# Autodesk Inventor assembly: Frame Test V3
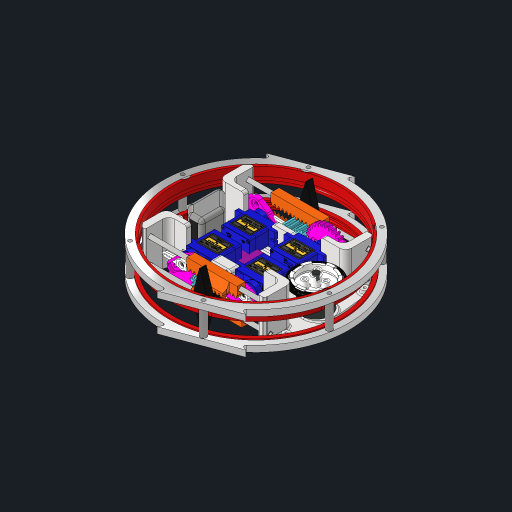
[picture p0: Inventor's stored thumbnail of the model, 512x512]
Saved by Autodesk Inventor 2023.2 (Build 272271030, 271C)
## iProperties
Created: 2024-01-27
Part Number: Frame Test V3
Document SubType Name: Assembly
Designer: robpl
Author: robpl
## Documents named in this file (17)
- C:\Users\robpl\OneDrive\Documents\Arduino\Onslaught\CAD\Onslaught V1.iam
- C:\Users\robpl\OneDrive\Documents\Arduino\Onslaught\CAD\Frame.ipt
- C:\Users\robpl\OneDrive\Documents\Arduino\Onslaught\CAD\SG90 - Micro Servo 9g - Tower Pro\SG90 - Micro Servo 9g - Tower Pro.ipt
- C:\Users\robpl\OneDrive\Documents\Arduino\Onslaught\CAD\802035 Battery.ipt
- C:\Users\robpl\OneDrive\Documents\Arduino\Onslaught\CAD\Ar620.ipt
- C:\Users\robpl\OneDrive\Documents\Arduino\Onslaught\CAD\Emax 1806 2280kv.ipt
- C:\Users\robpl\OneDrive\Documents\Arduino\Onslaught\CAD\BLHeli 12A ESC.ipt
- C:\Users\robpl\OneDrive\Documents\Arduino\Onslaught\CAD\Frame Test\Frame Test V3\Design Accelerator\Spur Gears3.iam
- C:\Users\robpl\OneDrive\Documents\Arduino\Onslaught\CAD\Frame Test\Servo Gear v3.ipt
- C:\Users\robpl\OneDrive\Documents\Arduino\Onslaught\CAD\Frame Test\Idler Gear.ipt
- C:\Users\robpl\OneDrive\Documents\Arduino\Onslaught\CAD\Frame Test\Rail.ipt
- C:\Users\robpl\OneDrive\Documents\Arduino\Onslaught\CAD\Frame Test\Rack V3.ipt
- C:\Users\robpl\OneDrive\Documents\Arduino\Onslaught\CAD\Frame Test\Leg V3.ipt
- C:\Users\robpl\OneDrive\Documents\Arduino\Onslaught\CAD\tamiya-slim-tire-set-1.snapshot.2\36mm Slim Tamiya.iam
- C:\Users\robpl\OneDrive\Documents\Arduino\Onslaught\CAD\2x6x2.5mm Bearing.ipt
- C:\Users\robpl\OneDrive\Documents\Arduino\Onslaught\CAD\Bearing Spacer.ipt
- C:\Users\robpl\OneDrive\Documents\Arduino\Onslaught\CAD\Frame Test\Ring.iam
## Components (35 placed, 16 different names)
1. Frame:1 — Mate:2, Mate:3, Mate:4, Mate:5, Mate:6, Mate:8, Mate:12, Mate:15, Mate:16, Mate:25, Angle:1, Angle:2, Angle:3, Angle:4, Flush:13, Flush:14, Mate:53, Mate:54, Mate:55, Mate:56, Mate:57, Mate:58, Mate:59, Mate:60, Mate:61, Mate:62, Mate:63, Mate:64, Flush:19, Flush:20, Mate:67, Mate:68, Flush:21, Mate:69, Mate:73, Mate:74, Mate:75, Mate:76, Flush:22, Mate:78, Mate:79, Mate:80, Mate:81, Mate:82, Mate:83, Mate:85
2. SG90 - Micro Servo 9g - Tower Pro:1 — Mate:15, Mate:16, Mate:29, Mate:32, Mate:55
3. SG90 - Micro Servo 9g - Tower Pro:2 — Mate:2, Mate:3, Mate:30, Mate:31, Mate:56, Mate:84
4. SG90 - Micro Servo 9g - Tower Pro:3 — Mate:4, Mate:8, Flush:10, Mate:24, Mate:54
5. SG90 - Micro Servo 9g - Tower Pro:4 — Mate:5, Mate:6, Mate:23, Flush:9, Mate:27, Mate:28, Mate:53
6. 802035 Battery:1 — Flush:6
7. 802035 Battery:2 — Flush:6
8. Ar620:1 — Mate:67, Mate:68, Flush:21
9. Emax 1806 2280kv:1 — Mate:12, Mate:21, Mate:65, Mate:66, Mate:82
10. BLHeli 12A ESC:1 — Mate:79
11. Spur Gears:2 [sub-assembly] — Mate:23, Flush:9
12. Servo Gear v3:1 — Flush:10, Mate:24
13. Idler Gear:1 — Mate:25, Flush:16
14. Servo Gear v3:2 — Mate:30, Mate:31
15. Servo Gear v3:3 — Mate:27, Mate:28
16. Servo Gear v3:4 — Mate:29, Mate:32
17. Rail:1 — Angle:1, Flush:14, Mate:62
18. Rail:2 — Angle:2, Flush:13, Mate:61
19. Rail:3 — Angle:4, Mate:63, Flush:19
20. Rail:4 — Angle:3, Mate:64, Flush:20
21. Rack V3:1 — Flush:18, Mate:51, Mate:52, Mate:58
22. Rack V3:2 — Flush:17, Mate:49, Mate:50, Mate:60
23. Rack V3:3 — Flush:17, Mate:59
24. Idler Gear:2 — Flush:16, Mate:85
25. Idler Gear:3 — Flush:15
26. Idler Gear:4 — Flush:15, Mate:83, Mate:84
27. Rack V3:4 — Flush:18, Mate:57
28. Leg V3:1 — Mate:49, Mate:50
29. Leg V3:2 — Mate:51, Mate:52
30. 36mm Slim Tamiya:1 [sub-assembly] — Mate:65, Mate:66
31. 2x6x2.5mm Bearing:1 — Mate:70, Mate:71
32. Bearing Spacer:1 — Mate:69, Mate:70, Mate:71, Mate:80, Mate:81
33. 2x6x2.5mm Bearing:2 — Mate:73, Mate:76
34. 2x6x2.5mm Bearing:3 — Mate:74, Mate:75
35. Ring:1 [sub-assembly] — Flush:22, Mate:78
## Relationships (71: Mate 54, Flush 13, Angle 4)
- Flush:6: 802035 Battery:1 ↔ 802035 Battery:2
- Mate:2: Frame:1 ↔ SG90 - Micro Servo 9g - Tower Pro:2
- Mate:3: Frame:1 ↔ SG90 - Micro Servo 9g - Tower Pro:2
- Mate:4: Frame:1 ↔ SG90 - Micro Servo 9g - Tower Pro:3
- Mate:5: Frame:1 ↔ SG90 - Micro Servo 9g - Tower Pro:4
- Mate:6: Frame:1 ↔ SG90 - Micro Servo 9g - Tower Pro:4
- Mate:8: Frame:1 ↔ SG90 - Micro Servo 9g - Tower Pro:3
- Mate:12 (1 mm): Frame:1 ↔ Emax 1806 2280kv:1
- Mate:15: Frame:1 ↔ SG90 - Micro Servo 9g - Tower Pro:1
- Mate:16: Frame:1 ↔ SG90 - Micro Servo 9g - Tower Pro:1
- Mate:21: Emax 1806 2280kv:1
- Mate:23: SG90 - Micro Servo 9g - Tower Pro:4 ↔ Spur Gears:2
- Flush:9: SG90 - Micro Servo 9g - Tower Pro:4 ↔ Spur Gears:2
- Flush:10: SG90 - Micro Servo 9g - Tower Pro:3 ↔ Servo Gear v3:1
- Mate:24: SG90 - Micro Servo 9g - Tower Pro:3 ↔ Servo Gear v3:1
- Mate:25: Frame:1 ↔ Idler Gear:1
- Mate:27: SG90 - Micro Servo 9g - Tower Pro:4 ↔ Servo Gear v3:3
- Mate:28: SG90 - Micro Servo 9g - Tower Pro:4 ↔ Servo Gear v3:3
- Mate:29: SG90 - Micro Servo 9g - Tower Pro:1 ↔ Servo Gear v3:4
- Mate:30: SG90 - Micro Servo 9g - Tower Pro:2 ↔ Servo Gear v3:2
- Mate:31: SG90 - Micro Servo 9g - Tower Pro:2 ↔ Servo Gear v3:2
- Mate:32: SG90 - Micro Servo 9g - Tower Pro:1 ↔ Servo Gear v3:4
- Angle:1 (0 deg): Frame:1 ↔ Rail:1
- Angle:2 (0 deg): Frame:1 ↔ Rail:2
- Angle:3 (0 deg): Frame:1 ↔ Rail:4
- Angle:4 (0 deg): Frame:1 ↔ Rail:3
- Flush:13: Frame:1 ↔ Rail:2
- Flush:14: Frame:1 ↔ Rail:1
- Flush:15: Idler Gear:3 ↔ Idler Gear:4
- Flush:16: Idler Gear:1 ↔ Idler Gear:2
- Flush:17: Rack V3:2 ↔ Rack V3:3
- Flush:18: Rack V3:1 ↔ Rack V3:4
- Mate:49 (-4.75 mm): Rack V3:2 ↔ Leg V3:1
- Mate:50 (-13.5 mm): Rack V3:2 ↔ Leg V3:1
- Mate:51 (-4.75 mm): Rack V3:1 ↔ Leg V3:2
- Mate:52 (-13.5 mm): Rack V3:1 ↔ Leg V3:2
- Mate:53: Frame:1 ↔ SG90 - Micro Servo 9g - Tower Pro:4
- Mate:54: Frame:1 ↔ SG90 - Micro Servo 9g - Tower Pro:3
- Mate:55: Frame:1 ↔ SG90 - Micro Servo 9g - Tower Pro:1
- Mate:56: Frame:1 ↔ SG90 - Micro Servo 9g - Tower Pro:2
- Mate:57: Frame:1 ↔ Rack V3:4
- Mate:58: Frame:1 ↔ Rack V3:1
- Mate:59: Frame:1 ↔ Rack V3:3
- Mate:60: Frame:1 ↔ Rack V3:2
- Mate:61: Frame:1 ↔ Rail:2
- Mate:62: Frame:1 ↔ Rail:1
- Mate:63: Frame:1 ↔ Rail:3
- Mate:64: Frame:1 ↔ Rail:4
- Flush:19: Frame:1 ↔ Rail:3
- Flush:20: Frame:1 ↔ Rail:4
- Mate:65: Emax 1806 2280kv:1 ↔ 36mm Slim Tamiya:1
- Mate:66: Emax 1806 2280kv:1 ↔ 36mm Slim Tamiya:1
- Mate:67: Frame:1 ↔ Ar620:1
- Mate:68: Frame:1 ↔ Ar620:1
- Flush:21: Frame:1 ↔ Ar620:1
- Mate:69: Frame:1 ↔ Bearing Spacer:1
- Mate:70: 2x6x2.5mm Bearing:1 ↔ Bearing Spacer:1
- Mate:71: 2x6x2.5mm Bearing:1 ↔ Bearing Spacer:1
- Mate:73: Frame:1 ↔ 2x6x2.5mm Bearing:2
- Mate:74: Frame:1 ↔ 2x6x2.5mm Bearing:3
- Mate:75: Frame:1 ↔ 2x6x2.5mm Bearing:3
- Mate:76: Frame:1 ↔ 2x6x2.5mm Bearing:2
- Flush:22 (-2.5 mm): Frame:1 ↔ Ring:1
- Mate:78: Frame:1 ↔ Ring:1
- Mate:79: Frame:1 ↔ BLHeli 12A ESC:1
- Mate:80: Frame:1 ↔ Bearing Spacer:1
- Mate:81: Frame:1 ↔ Bearing Spacer:1
- Mate:82: Frame:1 ↔ Emax 1806 2280kv:1
- Mate:83 (0.5 mm): Frame:1 ↔ Idler Gear:4
- Mate:84: SG90 - Micro Servo 9g - Tower Pro:2 ↔ Idler Gear:4
- Mate:85: Frame:1 ↔ Idler Gear:2
